# Autodesk Inventor assembly: reducer_1_MIR
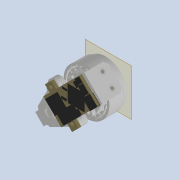
[picture p0: Inventor's stored thumbnail of the model, 180x180]
Saved by Autodesk Inventor 2023 (Build 270158000, 158)
## iProperties
Created: 2020-12-06
Part Number: reducer_1_MIR
Document SubType Name: Assembly
Designer: Shuang Peng
Author: Shuang Peng
## Documents named in this file (9)
- D:\projects-3\biped_tiny\hardware\reducer_1_MIR.iam
- D:\projects-3\biped_tiny\hardware\mot_27_ass_MIR.iam
- D:\projects-3\biped_tiny\hardware\tendon_wh_1_MIR.ipt
- D:\projects-3\biped_tiny\hardware\mot_holder_1_MIR.ipt
- D:\projects-3\biped_tiny\hardware\bearing_3_6_2_MIR.ipt
- D:\projects-3\biped_tiny\hardware\pin_3_15_MIR.ipt
- D:\projects-3\biped_tiny\hardware\screw_holder_2_3_MIR.ipt
- D:\projects-3\biped_tiny\hardware\encoder_holder_2_MIR.ipt
- D:\projects-3\biped_tiny\hardware\eletronic\brushless sub driver 2 v1\brushless sub driver 2_MIR.iam
## Components (13 placed, 8 different names)
1. mot_27_ass_MIR:1 [sub-assembly] — Insert:2, Insert:1, Flush:1, Insert:4, Insert:3, Flush:2
2. tendon_wh_1_MIR:1 — Insert:2, Insert:1, Flush:1, Flush:3
3. mot_holder_1_MIR:1 — Insert:4, Insert:3, Flush:2, Insert:5, Insert:16, Insert:14, Insert:15, Insert:19, Insert:18, Flush:4, Insert:29, Insert:28
4. bearing_3_6_2_MIR:1 — Insert:5
5. bearing_3_6_2_MIR:2 — Insert:16, Insert:8
6. pin_3_15_MIR:1 — Insert:8
7. screw_holder_2_3_MIR:1 — Insert:14
8. screw_holder_2_3_MIR:2 — Insert:15
9. encoder_holder_2_MIR:1 — Insert:19, Insert:18, Flush:4, Insert:17, Insert:21
10. screw_holder_2_3_MIR:3 — Insert:17, Insert:20
11. brushless sub driver 2_MIR:1 [sub-assembly] — Insert:21, Insert:20
12. screw_holder_2_3_MIR:4 — Insert:29
13. screw_holder_2_3_MIR:5 — Insert:28
## Relationships (20: Insert 16, Mate 3, Flush 1)
- Insert:2: mot_27_ass_MIR:1 ↔ tendon_wh_1_MIR:1
- Insert:1: mot_27_ass_MIR:1 ↔ tendon_wh_1_MIR:1
- Flush:1 [Mate]: mot_27_ass_MIR:1 ↔ tendon_wh_1_MIR:1
- Insert:4: mot_27_ass_MIR:1 ↔ mot_holder_1_MIR:1
- Insert:3: mot_27_ass_MIR:1 ↔ mot_holder_1_MIR:1
- Flush:2 [Mate]: mot_27_ass_MIR:1 ↔ mot_holder_1_MIR:1
- Insert:5: mot_holder_1_MIR:1 ↔ bearing_3_6_2_MIR:1
- Insert:16: mot_holder_1_MIR:1 ↔ bearing_3_6_2_MIR:2
- Flush:3 (1.5 mm): tendon_wh_1_MIR:1
- Insert:8: bearing_3_6_2_MIR:2 ↔ pin_3_15_MIR:1
- Insert:14: mot_holder_1_MIR:1 ↔ screw_holder_2_3_MIR:1
- Insert:15: mot_holder_1_MIR:1 ↔ screw_holder_2_3_MIR:2
- Insert:19: mot_holder_1_MIR:1 ↔ encoder_holder_2_MIR:1
- Insert:18: mot_holder_1_MIR:1 ↔ encoder_holder_2_MIR:1
- Flush:4 [Mate]: mot_holder_1_MIR:1 ↔ encoder_holder_2_MIR:1
- Insert:17: encoder_holder_2_MIR:1 ↔ screw_holder_2_3_MIR:3
- Insert:21: encoder_holder_2_MIR:1 ↔ brushless sub driver 2_MIR:1
- Insert:20: screw_holder_2_3_MIR:3 ↔ brushless sub driver 2_MIR:1
- Insert:29: mot_holder_1_MIR:1 ↔ screw_holder_2_3_MIR:4
- Insert:28: mot_holder_1_MIR:1 ↔ screw_holder_2_3_MIR:5
